# Autodesk Inventor assembly: spoolass
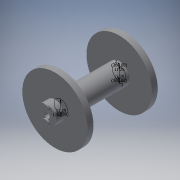
[picture p0: Inventor's stored thumbnail of the model, 180x180]
Saved by Autodesk Inventor 2017 (Build 210142000, 142)
## iProperties
Created: 2017-04-29
Part Number: spoolass
Document SubType Name: Assembly
Designer: s4321966
Author: s4321966
## Documents named in this file (4)
- \\puffball.labs.eait.uq.edu.au\s4321966\Documents\metr4810_spool draft\PARTS\spoolass.iam
- \\puffball.labs.eait.uq.edu.au\s4321966\Documents\metr4810_spool draft\PARTS\bolt.ipt
- \\puffball.labs.eait.uq.edu.au\s4321966\Documents\metr4810_spool draft\PARTS\Spool.ipt
- \\puffball.labs.eait.uq.edu.au\s4321966\Documents\metr4810_spool draft\PARTS\Spool_shaft.ipt
## Components (7 placed, 3 different names)
1. bolt:1 — Mate:6, Tangent:1, Tangent:6
2. Spool:1 — Mate:1, Mate:5, Mate:6, Tangent:1, Tangent:2, Mate:8
3. Spool_shaft:1 — Mate:1, Mate:2, Mate:7, Mate:8, Tangent:5, Tangent:6, Tangent:7, Tangent:8
4. Spool:2 — Mate:2, Mate:3, Mate:4, Tangent:3, Tangent:4, Mate:7
5. bolt:2 — Mate:4, Tangent:4, Tangent:8
6. bolt:3 — Mate:3, Tangent:3, Tangent:7
7. bolt:4 — Mate:5, Tangent:2, Tangent:5
## Relationships (16: Mate 8, Tangent 8)
- Mate:1: Spool:1 ↔ Spool_shaft:1
- Mate:2: Spool_shaft:1 ↔ Spool:2
- Mate:3: Spool:2 ↔ bolt:3
- Mate:4: Spool:2 ↔ bolt:2
- Mate:5: Spool:1 ↔ bolt:4
- Mate:6: bolt:1 ↔ Spool:1
- Tangent:1: bolt:1 ↔ Spool:1
- Tangent:2: Spool:1 ↔ bolt:4
- Tangent:3: Spool:2 ↔ bolt:3
- Tangent:4: Spool:2 ↔ bolt:2
- Mate:7: Spool_shaft:1 ↔ Spool:2
- Mate:8: Spool:1 ↔ Spool_shaft:1
- Tangent:5: Spool_shaft:1 ↔ bolt:4
- Tangent:6: bolt:1 ↔ Spool_shaft:1
- Tangent:7: Spool_shaft:1 ↔ bolt:3
- Tangent:8: Spool_shaft:1 ↔ bolt:2
